# Autodesk Inventor assembly: 組合4-15
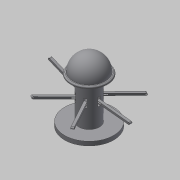
[picture p0: Inventor's stored thumbnail of the model, 180x180]
Saved by Autodesk Inventor 2018 (Build 220112000, 112)
## iProperties
Created: 2021-04-15
Part Number: 組合4-15
Material: 一般
Document SubType Name: Assembly
Designer: 王鼎鈞
Author: 王鼎鈞
## Documents named in this file (5)
- D:\2021顏家民\四人圖檔\組合4-15.iam
- D:\2021顏家民\四人圖檔\3d凸輪4-15.ipt
- D:\2021顏家民\四人圖檔\支架4-15.ipt
- D:\2021顏家民\四人圖檔\支架滑塊4-15.ipt
- D:\2021顏家民\四人圖檔\主體4-15.ipt
## Components (14 placed, 4 different names)
1. 3d凸輪4-15:1 — 插入:2, 相切:1
2. 支架4-15:1 — 插入:1, 貼合:1, 貼合:2
3. 支架滑塊4-15:1 — 插入:1, 相切:1
4. 主體4-15:1 — 插入:2, 貼合:1, 貼合:2, 貼合:3, 貼合:4, 插入:8, 插入:9, 插入:10, 插入:11
5. 支架4-15:2 — 貼合:3, 貼合:4
6. 支架滑塊4-15:2
7. 支架4-15:3 — 插入:9
8. 支架滑塊4-15:3
9. 支架4-15:4 — 插入:8
10. 支架滑塊4-15:4
11. 支架4-15:5 — 插入:10
12. 支架滑塊4-15:5
13. 支架4-15:6 — 插入:11
14. 支架滑塊4-15:6
## Relationships (16: Insert 11, Mate 4, Tangent 1)
- 插入:1 [Insert]: 支架4-15:1 ↔ 支架滑塊4-15:1
- 插入:2 [Insert]: 3d凸輪4-15:1 ↔ 主體4-15:1
- 貼合:1 [Mate]: 支架4-15:1 ↔ 主體4-15:1
- 貼合:2 [Mate]: 支架4-15:1 ↔ 主體4-15:1
- 相切:1 [Tangent]: 3d凸輪4-15:1 ↔ 支架滑塊4-15:1
- [Insert]: 支架4-15:2 ↔ 支架滑塊4-15:2
- [Insert]: 支架4-15:3 ↔ 支架滑塊4-15:3
- [Insert]: 支架4-15:4 ↔ 支架滑塊4-15:4
- [Insert]: 支架4-15:5 ↔ 支架滑塊4-15:5
- [Insert]: 支架4-15:6 ↔ 支架滑塊4-15:6
- 貼合:3 [Mate]: 主體4-15:1 ↔ 支架4-15:2
- 貼合:4 [Mate]: 主體4-15:1 ↔ 支架4-15:2
- 插入:8 [Insert]: 主體4-15:1 ↔ 支架4-15:4
- 插入:9 [Insert]: 主體4-15:1 ↔ 支架4-15:3
- 插入:10 [Insert]: 主體4-15:1 ↔ 支架4-15:5
- 插入:11 [Insert]: 主體4-15:1 ↔ 支架4-15:6
## Named parameters: d5_d0 = 0 mm, d6_d0 = 0 mm, d7_d0 = 0 mm, d8_d0 = 0 mm, d9_d0 = 0 mm
